# Autodesk Inventor assembly: Rack_series
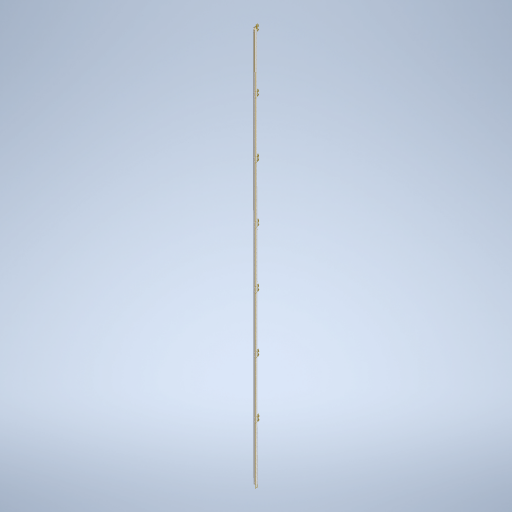
[picture p0: Inventor's stored thumbnail of the model, 512x512]
Saved by Autodesk Inventor 2023 (Build 270158000, 158)
## iProperties
Created: 2022-08-24
Part Number: Rack_series
Document SubType Name: Assembly
Designer: matte
Author: matte
## Documents named in this file (5)
- C:\Users\matte\Documents\GitHub\MDM-CyberOrto-CAD\Rack_Pinion\Rack_series_upper.iam
- C:\Users\matte\Documents\GitHub\MDM-CyberOrto-CAD\Rack_Pinion\Rack.ipt
- C:\Users\matte\Documents\GitHub\MDM-CyberOrto-CAD\Parker components\02-Fasteners\10-Standard T-Nuts\20-049.ipt
- C:\Users\matte\Documents\GitHub\MDM-CyberOrto-CAD\Rack_Pinion\Riduttore.ipt
- C:\Users\matte\Documents\GitHub\MDM-CyberOrto-CAD\Parker components\02-Fasteners\16-Screws\01-Metric Screws\03-Socket Head\24-320-4.ipt
## Components (42 placed, 4 different names)
1. Rack:1 — Coincidente:8, Coincidente:9, Angolo:1
2. Riduttore:1
3. 24-320-4:2 — Coincidente:9
4. 20-049:1 — Coincidente:8, Angolo:1
5. Riduttore:2
6. 24-320-4:1
7. Rack:2
8. Riduttore:3
9. 24-320-4:3
10. 20-049:2
11. Riduttore:4
12. 24-320-4:4
13. Rack:3
14. Riduttore:5
15. 24-320-4:5
16. 20-049:3
17. Riduttore:6
18. 24-320-4:6
19. Rack:4
20. Riduttore:7
21. 24-320-4:7
22. 20-049:4
23. Riduttore:8
24. 24-320-4:8
25. Rack:5
26. Riduttore:9
27. 24-320-4:9
28. 20-049:5
29. Riduttore:10
30. 24-320-4:10
31. Rack:6
32. Riduttore:11
33. 24-320-4:11
34. 20-049:6
35. Riduttore:12
36. 24-320-4:12
37. Rack:7
38. Riduttore:13
39. 24-320-4:13
40. 20-049:7
41. Riduttore:14
42. 24-320-4:14
## Component patterns: (7 elements, first: Rack:1 + Riduttore:1 + 24-320-4:2 + 20-049:1 + Riduttore:2 + 24-320-4:1)
## Relationships (11: Mate 9, Flush 1, Angle 1)
- [Mate]: Riduttore:1 ↔ 20-049:1
- [Mate]: Riduttore:1 ↔ 20-049:1
- [Mate]: 20-049:1 ↔ Riduttore:2
- [Mate]: 20-049:1 ↔ Riduttore:2
- [Mate]: Riduttore:2 ↔ 24-320-4:1
- [Mate]: Riduttore:1 ↔ 24-320-4:2
- [Flush]: 24-320-4:2 ↔ 24-320-4:1
- [Mate]: Rack:1 ↔ 24-320-4:2
- Coincidente:8 [Mate] (4.5 mm): Rack:1 ↔ 20-049:1
- Coincidente:9 [Mate]: Rack:1 ↔ 24-320-4:2
- Angolo:1 [Angle] (0 deg): Rack:1 ↔ 20-049:1
## Named parameters: d28_d25 = 0 mm, d29_d26 = 0 mm, d30_d27 = 0 mm, d31_d6 = 0 mm, d32_d7 = 0 mm, d33_d8 = 0 mm, d34_d9 = 0 mm, reps = 7
